# Autodesk Inventor assembly: Assembly
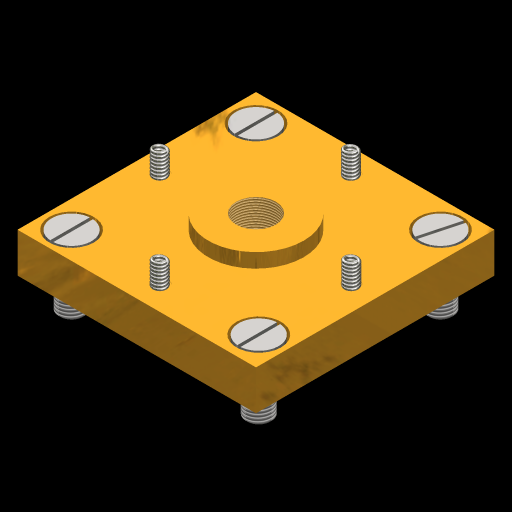
[picture p0: Inventor's stored thumbnail of the model, 512x512]
Saved by Autodesk Inventor 2024 (Build 280153000, 153)
## iProperties
Created: 2023-11-16
Part Number: Assembly
Document SubType Name: Assembly
Designer: Admin
Author: Admin
## Documents named in this file (11)
- C:\Users\Administrator\Documents\AUTODESK\Exercise\class7.assembly\Assembly.iam
- C:\Users\Administrator\Documents\AUTODESK\Exercise\class7.assembly\BasePlate.ipt
- C:\Users\Administrator\Documents\AUTODESK\Exercise\class7.assembly\M16bolt.ipt
- C:\Users\Administrator\Documents\AUTODESK\Exercise\class7.assembly\spring.ipt
- C:\Users\Administrator\Documents\AUTODESK\Exercise\class7.assembly\Body.ipt
- C:\Users\Administrator\Documents\AUTODESK\Exercise\class7.assembly\Stud.ipt
- C:\Users\Administrator\Documents\AUTODESK\Exercise\class7.assembly\ClampingNut.ipt
- C:\Users\Administrator\Documents\AUTODESK\Exercise\class7.assembly\Ball.ipt
- C:\Users\Administrator\Documents\AUTODESK\Exercise\class7.assembly\Handle.ipt
- C:\Users\Administrator\Documents\AUTODESK\Exercise\class7.assembly\Knob.ipt
- C:\Users\Administrator\Documents\AUTODESK\Exercise\class7.assembly\SetScrew.ipt
## Components (23 placed, 10 different names)
1. BasePlate:1 — Mate:1, Mate:2, Mate:3, Mate:4, Flush:1, Flush:2, Flush:3, Flush:4, Flush:6, Flush:7, Flush:8, Flush:9, Mate:13, Tangent:2, Mate:16, Flush:15, Mate:25
2. M16bolt:1 — Mate:1, Flush:4
3. M16bolt:2 — Mate:2, Flush:1
4. M16bolt:3 — Mate:3, Flush:2
5. M16bolt:4 — Mate:4, Flush:3
6. spring:1 — Flush:8, Mate:11, Mate:12
7. spring:2 — Mate:6, Flush:7, Mate:7
8. spring:3 — Mate:5, Flush:6, Mate:8, Tangent:1
9. spring:4 — Flush:9, Mate:9, Mate:10
10. Body:1 — Mate:13, Tangent:1, Mate:14, Tangent:2, Mate:16, Tangent:3, Mate:17, Mate:21, Mate:22, Mate:23, Mate:24
11. Stud:1 — Mate:14, Tangent:3, Flush:15, Mate:18
12. ClampingNut:1 — Mate:17, Mate:18, Insert:1
13. Handle:1 — Insert:1, Mate:19, Mate:20
14. Knob:1 — Mate:19, Mate:20
15. Ball:1 — Mate:25
16. SetScrew:1 — Mate:21, Mate:22
17. SetScrew:2
18. SetScrew:3
19. SetScrew:4
20. SetScrew:5 — Mate:23, Mate:24
21. SetScrew:6
22. SetScrew:7
23. SetScrew:8
## Component patterns: (4 elements, first: SetScrew:1), (4 elements, first: SetScrew:5)
## Relationships (43: Mate 24, Flush 15, Tangent 3, Insert 1)
- Mate:1: BasePlate:1 ↔ M16bolt:1
- Mate:2: BasePlate:1 ↔ M16bolt:2
- Mate:3: BasePlate:1 ↔ M16bolt:3
- Mate:4: BasePlate:1 ↔ M16bolt:4
- Flush:1: BasePlate:1 ↔ M16bolt:2
- Flush:2: BasePlate:1 ↔ M16bolt:3
- Flush:3: BasePlate:1 ↔ M16bolt:4
- Flush:4: BasePlate:1 ↔ M16bolt:1
- Flush:5 (-7.5 mm)
- Mate:5: spring:3
- Mate:6: spring:2
- Flush:6: BasePlate:1 ↔ spring:3
- Flush:7: BasePlate:1 ↔ spring:2
- Flush:8: BasePlate:1 ↔ spring:1
- Flush:9: BasePlate:1 ↔ spring:4
- Flush:10 (-51.25 mm)
- Mate:7: spring:2
- Flush:11 (69.25 mm)
- Flush:12 (9 mm)
- Flush:13 (52.75 mm)
- Flush:14 (-67.5 mm)
- Mate:8: spring:3
- Mate:9: spring:4
- Mate:10: spring:4
- Mate:11: spring:1
- Mate:12: spring:1
- Mate:13: BasePlate:1 ↔ Body:1
- Tangent:1: spring:3 ↔ Body:1
- Mate:14: Body:1 ↔ Stud:1
- Tangent:2: BasePlate:1 ↔ Body:1
- Mate:16 (1 mm): BasePlate:1 ↔ Body:1
- Tangent:3: Body:1 ↔ Stud:1
- Flush:15: BasePlate:1 ↔ Stud:1
- Mate:17: Body:1 ↔ ClampingNut:1
- Mate:18: Stud:1 ↔ ClampingNut:1
- Insert:1: ClampingNut:1 ↔ Handle:1
- Mate:19: Handle:1 ↔ Knob:1
- Mate:20: Handle:1 ↔ Knob:1
- Mate:21: Body:1 ↔ SetScrew:1
- Mate:22: Body:1 ↔ SetScrew:1
- Mate:23: Body:1 ↔ SetScrew:5
- Mate:24: Body:1 ↔ SetScrew:5
- Mate:25: BasePlate:1 ↔ Ball:1
